# Autodesk Inventor assembly: Full Car Assembly
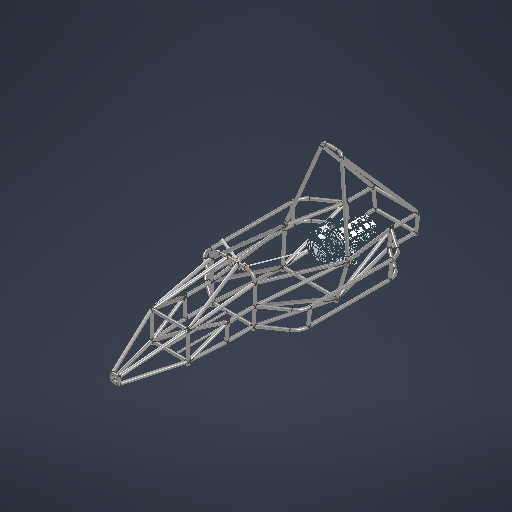
[picture p0: Inventor's stored thumbnail of the model, 512x512]
Saved by Autodesk Inventor 2026.1 (Build 301233000, 233)
## iProperties
Created: 2026-07-07
Part Number: Full Car Assembly
Document SubType Name: Assembly
Designer: share
Author: share
## Documents named in this file (15)
- C:\Users\share\OneDrive\Documents\Personal Projects\GOGO Kart\CAD\GOGO_KART_FSAE\Full Car Assembly.iam
- C:\Users\share\OneDrive\Documents\Personal Projects\GOGO Kart\CAD\GOGO_KART_FSAE\FrameV2\Frame\Frame 1780692296746.iam
- C:\Users\share\OneDrive\Documents\Personal Projects\GOGO Kart\CAD\GOGO_KART_FSAE\honda-cbr600-f4i-engine-1.snapshot.3\Honda CBR600 F4i\Honda CBR600 F4i\Honda CBR600 F4i.ipt
- C:\Users\share\OneDrive\Documents\Personal Projects\GOGO Kart\CAD\GOGO_KART_FSAE\Shifter\crank.ipt
- C:\Users\share\OneDrive\Documents\Personal Projects\GOGO Kart\CAD\GOGO_KART_FSAE\Shifter\59935K71_Ball Joint Rod End\59935K71_Ball Joint Rod End\59935K71_Ball Joint Rod End.ipt
- C:\Users\share\OneDrive\Documents\Personal Projects\GOGO Kart\CAD\GOGO_KART_FSAE\Shifter\threadedtubeshort.ipt
- C:\Users\share\OneDrive\Documents\Personal Projects\GOGO Kart\CAD\GOGO_KART_FSAE\Shifter\ShifterBracket.ipt
- C:\Users\share\OneDrive\Documents\Personal Projects\GOGO Kart\CAD\GOGO_KART_FSAE\Shifter\BellCrank.ipt
- C:\Users\share\OneDrive\Documents\Personal Projects\GOGO Kart\CAD\GOGO_KART_FSAE\Shifter\Bearing.ipt
- C:\Users\share\OneDrive\Documents\Personal Projects\GOGO Kart\CAD\GOGO_KART_FSAE\Shifter\spacer.ipt
- C:\Users\share\OneDrive\Documents\Personal Projects\GOGO Kart\CAD\GOGO_KART_FSAE\Shifter\6045N121_Low-Carbon Steel Round Tube\6045N121_Low-Carbon Steel Round Tube\6045N121_Low-Carbon Steel Round Tube.ipt
- C:\Users\share\OneDrive\Documents\Inventor\Content Center Files\R2026\en-US\ISO 4032(2)\ISO 4032 - M5 - ISO.ipt
- C:\Users\share\OneDrive\Documents\Personal Projects\GOGO Kart\CAD\GOGO_KART_FSAE\Rod Ends\5-8 Rod End Assembly.iam
- C:\Users\share\OneDrive\Documents\Personal Projects\GOGO Kart\CAD\GOGO_KART_FSAE\Shifter\stickshift.ipt
- C:\Users\share\OneDrive\Documents\Personal Projects\GOGO Kart\CAD\GOGO_KART_FSAE\Shifter\stickplate.ipt
## Components (18 placed, 14 different names)
1. Frame 1780692296746:1 [sub-assembly] — Flush:1, Flush:2, Flush:3, Engine Up Down Mate, Engine Sideways Mate, Tangent:1, Tangent:2
2. Honda CBR600 F4i:1 — Engine Up Down Mate, Engine Sideways Mate, Insert:1
3. crank:1 — Insert:1, Insert:2
4. 59935K71_Ball Joint Rod End:1 — Rotational:2, Angle:1, Rotational:6
5. 59935K71_Ball Joint Rod End:3 — Insert:2, Rotational:1, Angle:1
6. threadedtubeshort:1 — Rotational:1, Rotational:2
7. ShifterBracket:1 — Rigid:1, Tangent:1
8. BellCrank:1 — Rotational:3, Rotational:6, Insert:3
9. Bearing:1 — Rotational:3, Rotational:4, Rotational:5
10. spacer:1 — Rigid:1, Rotational:4
11. spacer:2 — Rotational:5
12. 6045N121_Low-Carbon Steel Round Tube:1 — Rigid:2, Rigid:3
13. ISO 4032 M5:1 — Rigid:3, Rotational:8
14. ISO 4032 M5:2 — Rigid:2, Rotational:7
15. 5-8 Rod End Assembly:1 [sub-assembly] — Rotational:8, Rotational:9
16. 5-8 Rod End Assembly:2 [sub-assembly] — Rotational:7, Insert:3
17. stickshift:1 — Rigid:4, Rotational:9
18. stickplate:1 — Rigid:4, Tangent:2
## Relationships (24: RevoluteJoint 9, Flush 5, WeldJoint 4, Insert 3, Tangent 2, Angle 1)
- Flush:1 (428.457 mm): Frame 1780692296746:1
- Flush:2 (-681.212 mm): Frame 1780692296746:1
- Flush:3 (-922.539 mm): Frame 1780692296746:1
- Engine Up Down Mate [Flush] (-300 mm): Frame 1780692296746:1 ↔ Honda CBR600 F4i:1
- Engine Sideways Mate [Flush] (-40 mm): Frame 1780692296746:1 ↔ Honda CBR600 F4i:1
- Insert:1 (-5 mm): Honda CBR600 F4i:1 ↔ crank:1
- Insert:2: crank:1 ↔ 59935K71_Ball Joint Rod End:3
- Rotational:1 [RevoluteJoint]: 59935K71_Ball Joint Rod End:3 ↔ threadedtubeshort:1
- Rotational:2 [RevoluteJoint]: 59935K71_Ball Joint Rod End:1 ↔ threadedtubeshort:1
- Angle:1 (90 deg): 59935K71_Ball Joint Rod End:1 ↔ 59935K71_Ball Joint Rod End:3
- Rigid:1 [WeldJoint]: ShifterBracket:1 ↔ spacer:1
- Rotational:3 [RevoluteJoint]: BellCrank:1 ↔ Bearing:1
- Rotational:4 [RevoluteJoint]: Bearing:1 ↔ spacer:1
- Rotational:5 [RevoluteJoint]: Bearing:1 ↔ spacer:2
- Rotational:6 [RevoluteJoint]: 59935K71_Ball Joint Rod End:1 ↔ BellCrank:1
- Tangent:1: Frame 1780692296746:1 ↔ ShifterBracket:1
- Rigid:2 [WeldJoint]: 6045N121_Low-Carbon Steel Round Tube:1 ↔ ISO 4032 M5:2
- Rigid:3 [WeldJoint]: 6045N121_Low-Carbon Steel Round Tube:1 ↔ ISO 4032 M5:1
- Rotational:7 [RevoluteJoint]: ISO 4032 M5:2 ↔ 5-8 Rod End Assembly:2
- Insert:3: BellCrank:1 ↔ 5-8 Rod End Assembly:2
- Rotational:8 [RevoluteJoint]: ISO 4032 M5:1 ↔ 5-8 Rod End Assembly:1
- Rigid:4 [WeldJoint]: stickshift:1 ↔ stickplate:1
- Tangent:2: Frame 1780692296746:1 ↔ stickplate:1
- Rotational:9 [RevoluteJoint]: 5-8 Rod End Assembly:1 ↔ stickshift:1
